# Autodesk Inventor assembly: Clutch Assembly
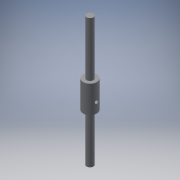
[picture p0: Inventor's stored thumbnail of the model, 180x180]
Saved by Autodesk Inventor 2016 (Build 200138000, 138)
## iProperties
Created: 2015-06-15
Part Number: Clutch Assembly
Document SubType Name: Assembly
Designer: steele
Author: steele
## Documents named in this file (3)
- C:\snobotics\CAD\robSteele\Bevel Gearbox\2015 Summer Bevel Gearbox\Clutch Assembly.iam
- C:\snobotics\CAD\robSteele\Bevel Gearbox\2015 Summer Bevel Gearbox\Part of Clutch.ipt
- C:\snobotics\CAD\robSteele\Bevel Gearbox\2015 Summer Bevel Gearbox\Lower Half of Clutch.ipt
## Components (2 placed, 2 different names)
1. Part of Clutch:1 — Insert:1
2. Lower Half of Clutch:1 — Insert:1
## Relationships (1: Insert 1)
- Insert:1: Part of Clutch:1 ↔ Lower Half of Clutch:1
